# Autodesk Inventor assembly: WasabiV2
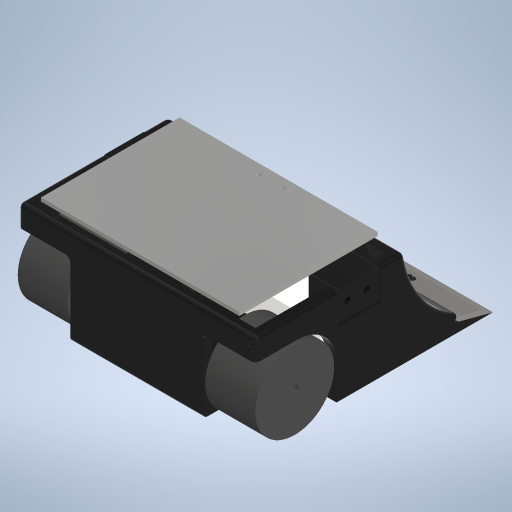
[picture p0: Inventor's stored thumbnail of the model, 512x512]
Saved by Autodesk Inventor 2024 (Build 280153000, 153)
## iProperties
Created: 2024-03-09
Part Number: WasabiV2
Document SubType Name: Assembly
Designer: kdcao
Author: kdcao
## Documents named in this file (9)
- C:\Users\kdcao\Documents\GitHub\wasabi2\Wasabi\WasabiV2.iam
- C:\Users\kdcao\Documents\GitHub\wasabi2\Wasabi\Body\bodyb2.ipt
- C:\Users\kdcao\Documents\GitHub\wasabi2\Wasabi\Bladev2.ipt
- C:\Users\kdcao\Documents\GitHub\wasabi2\Wasabi\Parts\micro-metal-gearmotor-standard.ipt
- C:\Users\kdcao\Documents\GitHub\wasabi2\Wasabi\Parts\wheel.ipt
- C:\Users\kdcao\Documents\GitHub\wasabi2\Wasabi\Parts\qtr-1a-reflectance-sensor.ipt
- C:\Users\kdcao\Documents\GitHub\wasabi2\Wasabi\Batteryv2.ipt
- C:\Users\kdcao\Documents\GitHub\wasabi2\Wasabi\pcb.ipt
- C:\Users\kdcao\Documents\GitHub\wasabi2\Wasabi\Parts\IR sensor.ipt
## Components (15 placed, 8 different names)
1. bodyb2:1 — Rigid:1, Rigid:2, Rigid:3, Rigid:4, Rigid:5, Rigid:6, Mate:1, Mate:2, Mate:3, Rigid:7, Rigid:8, Rigid:9, Mate:4, Mate:5, Mate:6, Mate:7, Mate:8
2. Bladev2:1 — Rigid:6
3. micro-metal-gearmotor-standard:1 — Rigid:2, Cylindrical:2
4. micro-metal-gearmotor-standard:2 — Rigid:1, Cylindrical:1
5. wheel:1 — Cylindrical:2
6. wheel:2 — Cylindrical:1
7. qtr-1a-reflectance-sensor:1 — Rigid:3
8. qtr-1a-reflectance-sensor:2 — Rigid:4
9. Batteryv2:1 — Rigid:5
10. pcb:1 — Mate:1, Mate:2, Mate:3
11. IR sensor:1 — Rigid:7
12. IR sensor:2 — Mate:4, Mate:5
13. IR sensor:3 — Rigid:8
14. IR sensor:4 — Rigid:9
15. IR sensor:5 — Mate:6, Mate:7, Mate:8
## Relationships (19: WeldJoint 9, Mate 8, CylindricalJoint 2)
- Rigid:1 [WeldJoint]: bodyb2:1 ↔ micro-metal-gearmotor-standard:2
- Rigid:2 [WeldJoint]: bodyb2:1 ↔ micro-metal-gearmotor-standard:1
- Cylindrical:1: micro-metal-gearmotor-standard:2 ↔ wheel:2
- Cylindrical:2: micro-metal-gearmotor-standard:1 ↔ wheel:1
- Rigid:3 [WeldJoint]: bodyb2:1 ↔ qtr-1a-reflectance-sensor:1
- Rigid:4 [WeldJoint]: bodyb2:1 ↔ qtr-1a-reflectance-sensor:2
- Rigid:5 [WeldJoint]: bodyb2:1 ↔ Batteryv2:1
- Rigid:6 [WeldJoint]: bodyb2:1 ↔ Bladev2:1
- Mate:1: bodyb2:1 ↔ pcb:1
- Mate:2: bodyb2:1 ↔ pcb:1
- Mate:3: bodyb2:1 ↔ pcb:1
- Rigid:7 [WeldJoint]: bodyb2:1 ↔ IR sensor:1
- Rigid:8 [WeldJoint]: bodyb2:1 ↔ IR sensor:3
- Rigid:9 [WeldJoint]: bodyb2:1 ↔ IR sensor:4
- Mate:4: bodyb2:1 ↔ IR sensor:2
- Mate:5: bodyb2:1 ↔ IR sensor:2
- Mate:6: bodyb2:1 ↔ IR sensor:5
- Mate:7: bodyb2:1 ↔ IR sensor:5
- Mate:8: bodyb2:1 ↔ IR sensor:5
